# Autodesk Inventor assembly: Micro_Mate-N-Lok_TE-Connectivity_3mm_2x8_Male
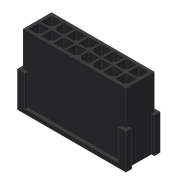
[picture p0: Inventor's stored thumbnail of the model, 180x180]
Saved by Autodesk Inventor 2015 (Build 190159000, 159)
## iProperties
Created: 2015-01-30
Part Number: Micro_Mate-N-Lok_TE-Connectivity_3mm_2x8_Male
Document SubType Name: Assembly
## Documents named in this file (3)
- C:\Dropbox\Inventor\Projects\001_EK-Teile\Micro_Mate-N-Lok_TE-Connectivity_3mm_2x8_Male.iam
- C:\Dropbox\Inventor\Projects\001_EK-Teile\Micro_Mate-N-Lok_TE-Connectivity_3mm_Crimp-Pin_1-794612-0.ipt
- C:\Dropbox\Inventor\Projects\001_EK-Teile\Micro_Mate-N-Lok_TE-Connectivity_3mm_2x8_Male_1-794616-6.ipt
## Components (17 placed, 2 different names)
1. Micro_Mate-N-Lok_TE-Connectivity_3mm_2x8_Male_1-794616-6:1 — Mate:3, Mate:2, Flush:3
2. Micro_Mate-N-Lok_TE-Connectivity_3mm_Crimp-Pin_1-794612-0:1 — Mate:3, Mate:2, Flush:3
3. Micro_Mate-N-Lok_TE-Connectivity_3mm_Crimp-Pin_1-794612-0:2
4. Micro_Mate-N-Lok_TE-Connectivity_3mm_Crimp-Pin_1-794612-0:3
5. Micro_Mate-N-Lok_TE-Connectivity_3mm_Crimp-Pin_1-794612-0:4
6. Micro_Mate-N-Lok_TE-Connectivity_3mm_Crimp-Pin_1-794612-0:5
7. Micro_Mate-N-Lok_TE-Connectivity_3mm_Crimp-Pin_1-794612-0:6
8. Micro_Mate-N-Lok_TE-Connectivity_3mm_Crimp-Pin_1-794612-0:7
9. Micro_Mate-N-Lok_TE-Connectivity_3mm_Crimp-Pin_1-794612-0:8
10. Micro_Mate-N-Lok_TE-Connectivity_3mm_Crimp-Pin_1-794612-0:9
11. Micro_Mate-N-Lok_TE-Connectivity_3mm_Crimp-Pin_1-794612-0:10
12. Micro_Mate-N-Lok_TE-Connectivity_3mm_Crimp-Pin_1-794612-0:11
13. Micro_Mate-N-Lok_TE-Connectivity_3mm_Crimp-Pin_1-794612-0:12
14. Micro_Mate-N-Lok_TE-Connectivity_3mm_Crimp-Pin_1-794612-0:13
15. Micro_Mate-N-Lok_TE-Connectivity_3mm_Crimp-Pin_1-794612-0:14
16. Micro_Mate-N-Lok_TE-Connectivity_3mm_Crimp-Pin_1-794612-0:15
17. Micro_Mate-N-Lok_TE-Connectivity_3mm_Crimp-Pin_1-794612-0:16
## Component patterns: (16 elements, first: Micro_Mate-N-Lok_TE-Connectivity_3mm_Crimp-Pin_1-794612-0:1)
## Relationships (3: Mate 2, Flush 1)
- Mate:3 (1.05 mm): Micro_Mate-N-Lok_TE-Connectivity_3mm_2x8_Male_1-794616-6:1 ↔ Micro_Mate-N-Lok_TE-Connectivity_3mm_Crimp-Pin_1-794612-0:1
- Mate:2 (1.13 mm): Micro_Mate-N-Lok_TE-Connectivity_3mm_2x8_Male_1-794616-6:1 ↔ Micro_Mate-N-Lok_TE-Connectivity_3mm_Crimp-Pin_1-794612-0:1
- Flush:3 (2.26 mm): Micro_Mate-N-Lok_TE-Connectivity_3mm_2x8_Male_1-794616-6:1 ↔ Micro_Mate-N-Lok_TE-Connectivity_3mm_Crimp-Pin_1-794612-0:1
